# Autodesk Inventor assembly: bepf_platforma_polka_gorna
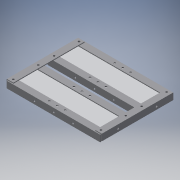
[picture p0: Inventor's stored thumbnail of the model, 180x180]
Saved by Autodesk Inventor 2017 (Build 210142000, 142)
## iProperties
Part Number: bepf_platforma_polka_gorna
Material: Ogólny
Document SubType Name: Assembly
Designer: gagato
Author: gagato
## Documents named in this file (4)
- C:\Users\gagato\Documents\bepf\bepf_platforma_polka_gorna.iam
- C:\Users\gagato\Documents\bepf\bepf_platforma_rama_bok_krotki.ipt
- C:\Users\gagato\Documents\bepf\bepf_platforma_rama_bok_dlugi.ipt
- C:\Users\gagato\Documents\bepf\bepf_platforma_wypelnienie_polka_gorna.ipt
## Components (8 placed, 3 different names)
1. bepf_platforma_rama_bok_krotki:1 — Zestawiający:1, Zestawiający:2, Zestawiający:3, Zestawiający:11, Zestawiający:15, Zestawiający:16, Zestawiający:18, Zestawiający:19, Symetria:2, Zestawiający:23, Zestawiający:24
2. bepf_platforma_rama_bok_krotki:2 — Zestawiający:4, Zestawiający:5, Zestawiający:10, Zestawiający:12, Zestawiający:13, Zestawiający:14, Zestawiający:17, Symetria:2
3. bepf_platforma_rama_bok_dlugi:1 — Zestawiający:17, Zestawiający:18, Zestawiający:19, Zestawiający:26
4. bepf_platforma_rama_bok_dlugi:2 — Zestawiający:14, Zestawiający:15, Zestawiający:16, Symetria:1, Zestawiający:21
5. bepf_platforma_rama_bok_dlugi:3 — Zestawiający:11, Zestawiający:12, Zestawiający:13, Symetria:1, Zestawiający:20, Zestawiający:25
6. bepf_platforma_rama_bok_dlugi:4 — Zestawiający:1, Zestawiający:2, Zestawiający:3, Zestawiający:4, Zestawiający:5, Zestawiający:10, Zestawiający:22
7. bepf_platforma_wypelnienie_polka_gorna:1 — Zestawiający:22, Zestawiający:23, Zestawiający:25
8. bepf_platforma_wypelnienie_polka_gorna:2 — Zestawiający:21, Zestawiający:24, Zestawiający:26
## Relationships (24: Mate 22, Symmetry 2)
- Zestawiający:1 [Mate]: bepf_platforma_rama_bok_krotki:1 ↔ bepf_platforma_rama_bok_dlugi:4
- Zestawiający:2 [Mate]: bepf_platforma_rama_bok_krotki:1 ↔ bepf_platforma_rama_bok_dlugi:4
- Zestawiający:3 [Mate]: bepf_platforma_rama_bok_krotki:1 ↔ bepf_platforma_rama_bok_dlugi:4
- Zestawiający:4 [Mate]: bepf_platforma_rama_bok_krotki:2 ↔ bepf_platforma_rama_bok_dlugi:4
- Zestawiający:5 [Mate]: bepf_platforma_rama_bok_krotki:2 ↔ bepf_platforma_rama_bok_dlugi:4
- Zestawiający:10 [Mate]: bepf_platforma_rama_bok_krotki:2 ↔ bepf_platforma_rama_bok_dlugi:4
- Zestawiający:11 [Mate]: bepf_platforma_rama_bok_krotki:1 ↔ bepf_platforma_rama_bok_dlugi:3
- Zestawiający:12 [Mate]: bepf_platforma_rama_bok_krotki:2 ↔ bepf_platforma_rama_bok_dlugi:3
- Zestawiający:13 [Mate]: bepf_platforma_rama_bok_krotki:2 ↔ bepf_platforma_rama_bok_dlugi:3
- Zestawiający:14 [Mate]: bepf_platforma_rama_bok_krotki:2 ↔ bepf_platforma_rama_bok_dlugi:2
- Zestawiający:15 [Mate]: bepf_platforma_rama_bok_krotki:1 ↔ bepf_platforma_rama_bok_dlugi:2
- Zestawiający:16 [Mate]: bepf_platforma_rama_bok_krotki:1 ↔ bepf_platforma_rama_bok_dlugi:2
- Zestawiający:17 [Mate]: bepf_platforma_rama_bok_krotki:2 ↔ bepf_platforma_rama_bok_dlugi:1
- Zestawiający:18 [Mate]: bepf_platforma_rama_bok_krotki:1 ↔ bepf_platforma_rama_bok_dlugi:1
- Zestawiający:19 [Mate]: bepf_platforma_rama_bok_krotki:1 ↔ bepf_platforma_rama_bok_dlugi:1
- Symetria:1 [Symmetry]: bepf_platforma_rama_bok_dlugi:2 ↔ bepf_platforma_rama_bok_dlugi:3
- Symetria:2 [Symmetry]: bepf_platforma_rama_bok_krotki:1 ↔ bepf_platforma_rama_bok_krotki:2
- Zestawiający:20 [Mate]: bepf_platforma_rama_bok_dlugi:3
- Zestawiający:21 [Mate]: bepf_platforma_rama_bok_dlugi:2 ↔ bepf_platforma_wypelnienie_polka_gorna:2
- Zestawiający:22 [Mate]: bepf_platforma_rama_bok_dlugi:4 ↔ bepf_platforma_wypelnienie_polka_gorna:1
- Zestawiający:23 [Mate]: bepf_platforma_rama_bok_krotki:1 ↔ bepf_platforma_wypelnienie_polka_gorna:1
- Zestawiający:24 [Mate]: bepf_platforma_rama_bok_krotki:1 ↔ bepf_platforma_wypelnienie_polka_gorna:2
- Zestawiający:25 [Mate]: bepf_platforma_rama_bok_dlugi:3 ↔ bepf_platforma_wypelnienie_polka_gorna:1
- Zestawiający:26 [Mate]: bepf_platforma_rama_bok_dlugi:1 ↔ bepf_platforma_wypelnienie_polka_gorna:2
